# Autodesk Inventor assembly: Milestone 2 Assembly
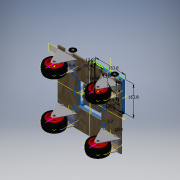
[picture p0: Inventor's stored thumbnail of the model, 180x180]
Saved by Autodesk Inventor 2016 (Build 200138000, 138)
## iProperties
Created: 2016-03-08
Part Number: Milestone 2 Assembly
Document SubType Name: Assembly
Designer: Kenneth Daniel
Author: Kenneth Daniel
## Documents named in this file (38)
- C:\Users\Kenneth Daniel\Documents\Enes 100A\Milestone 2\Milestone 2 Assembly.iam
- C:\Users\Kenneth Daniel\Documents\Enes 100A\Milestone 2\Lifting Platform With Balance.ipt
- C:\Users\Kenneth Daniel\Documents\Enes 100A\Milestone 2\To Much Work, Motor.ipt
- C:\Users\Kenneth Daniel\Documents\Enes 100A\Milestone One\PH Monitor.ipt
- C:\Users\Kenneth Daniel\Documents\Enes 100A\Milestone 2\Lifting Chasis Assembly Milestone 2.iam
- C:\Users\Kenneth Daniel\Documents\Enes 100A\Milestone 2\Lifting Motor Platform.ipt
- C:\Users\Kenneth Daniel\Documents\Enes 100A\Milestone 2\Milestone 2 Main Vehicle Chassis.ipt
- C:\Users\Kenneth Daniel\Documents\Enes 100A\arduino uno.iam
- C:\Users\Kenneth Daniel\Documents\Inventor\Content Center Files\R2016\en-US\AS 1427(00)\AS 1427 - M5 x 20(4).ipt
- C:\Users\Kenneth Daniel\Documents\Enes 100A\Milestone 2\Motors Mount For Chassis.ipt
- C:\Users\Kenneth Daniel\Documents\Enes 100A\CorrectMotor_CAD_spencermical_enes100OSVproject_4-50pm-3-3-16-thursday-freshmanyear-springsemester.ipt
- C:\Users\Kenneth Daniel\Documents\Enes 100A\Milestone 2\Updated Milestone 2 Wheel.ipt
- C:\Users\Kenneth Daniel\Documents\Enes 100A\Milestone 2\Milestone 2 Rim.ipt
- C:\Users\Kenneth Daniel\Documents\Enes 100A\Milestone 2\Small Sprocket.ipt
- C:\Users\Kenneth Daniel\Documents\Enes 100A\Milestone 2\Motors Mount For Chassis_MIR.ipt
- C:\Users\Kenneth Daniel\Documents\Enes 100A\CorrectMotor_CAD_spencermical_enes100OSVproject_4-50pm-3-3-16-thursday-freshmanyear-springsemester_MIR.ipt
- C:\Users\Kenneth Daniel\Documents\Enes 100A\Milestone 2\Motors Mount For Chassis_MIR2.ipt
- C:\Users\Kenneth Daniel\Documents\Enes 100A\CorrectMotor_CAD_spencermical_enes100OSVproject_4-50pm-3-3-16-thursday-freshmanyear-springsemester_MIR2.ipt
- C:\Users\Kenneth Daniel\Documents\Enes 100A\Milestone 2\Motors Mount For Chassis_MIR2_MIR.ipt
- C:\Users\Kenneth Daniel\Documents\Enes 100A\CorrectMotor_CAD_spencermical_enes100OSVproject_4-50pm-3-3-16-thursday-freshmanyear-springsemester_MIR2_MIR.ipt
- C:\Users\Kenneth Daniel\Documents\Enes 100A\Milestone 2\Small Sprocket_MIR.ipt
- C:\Users\Kenneth Daniel\Documents\Enes 100A\Milestone 2\Small Sprocket_MIR1.ipt
- C:\Users\Kenneth Daniel\Documents\Enes 100A\Milestone 2\Small Sprocket_MIR_MIR.ipt
- C:\Users\Kenneth Daniel\Documents\Inventor\Content Center Files\R2016\en-US\CNS 3128\CNS 3128 - M 5 x 0.8.ipt
- C:\Users\Kenneth Daniel\Documents\Enes 100A\Milestone 2\Wheel Holder Milestone 2.ipt
- C:\Users\Kenneth Daniel\Documents\Enes 100A\Milestone 2\Updated Milestone 2 Wheel_MIR6.ipt
- C:\Users\Kenneth Daniel\Documents\Enes 100A\Milestone 2\Milestone 2 Rim_MIR6.ipt
- C:\Users\Kenneth Daniel\Documents\Enes 100A\Milestone 2\Wheel Holder Milestone 2_MIR6.ipt
- C:\Users\Kenneth Daniel\Documents\Enes 100A\Milestone 2\Updated Milestone 2 Wheel_MIR7.ipt
- C:\Users\Kenneth Daniel\Documents\Enes 100A\Milestone 2\Milestone 2 Rim_MIR7.ipt
- C:\Users\Kenneth Daniel\Documents\Enes 100A\Milestone 2\Wheel Holder Milestone 2_MIR7.ipt
- C:\Users\Kenneth Daniel\Documents\Enes 100A\Milestone 2\Updated Milestone 2 Wheel_MIR6_MIR.ipt
- C:\Users\Kenneth Daniel\Documents\Enes 100A\Milestone 2\Milestone 2 Rim_MIR6_MIR.ipt
- C:\Users\Kenneth Daniel\Documents\Enes 100A\Milestone 2\Wheel Holder Milestone 2_MIR6_MIR.ipt
- C:\Users\Kenneth Daniel\Documents\Enes 100A\Simplistic_battery_pack-superdroid-spencermical.ipt
- C:\Users\Kenneth Daniel\Documents\Enes 100A\Syringe_moreaccurate_ENES100_OSV-spencermical-4-52pm-3-5-16-saturday.ipt
- C:\Users\Kenneth Daniel\Documents\Enes 100A\Larger Syringe.ipt
- C:\Users\Kenneth Daniel\Documents\Enes 100A\Vex Motor.iam
## Components (52 placed, 37 different names)
1. Lifting Platform With Balance:1 — Mate:8, Mate:9, Mate:10, Mate:11, Mate:18, Mate:19
2. To Much Work, Motor:1 — Mate:8, Mate:9
3. PH Monitor:1 — Mate:10, Mate:11
4. Lifting Chasis Assembly Milestone 2:1 [sub-assembly] — Mate:15, Mate:16, Mate:17, Mate:18, Mate:19, Mate:20, Mate:21, Mate:22, Mate:90
5. Lifting Motor Platform:1 — Mate:15, Mate:16, Mate:17, Mate:92, Angle:1, Mate:93, Flush:28
6. Milestone 2 Main Vehicle Chassis:1 — Mate:20, Mate:21, Mate:22, Mate:23, Mate:33, Mate:34, Mate:35, Mate:36, Flush:5, Mate:37, Flush:6, Mate:39, Mate:49, Mate:52, Mate:57, Mate:62, Mate:63, Mate:72, Mate:74, Mate:76, Mate:77, Mate:78, Mate:79, Flush:13, Flush:18, Flush:24, Flush:25, Flush:26, Flush:27, Mate:89, Tangent:1, Tangent:2, Mate:94, Mate:95
7. arduino uno:1 [sub-assembly] — Mate:33, Mate:34
8. AS 1427 - Metric M5 x 20:1 — Mate:50, Mate:51, Mate:57, Mate:73
9. AS 1427 - Metric M5 x 20:2 — Mate:55, Mate:56, Mate:71
10. AS 1427 - Metric M5 x 20:3 — Mate:60, Mate:61
11. AS 1427 - Metric M5 x 20:4 — Mate:58, Mate:59, Mate:62
12. AS 1427 - Metric M5 x 20:5 — Mate:53, Mate:54
13. AS 1427 - Metric M5 x 20:8 — Mate:47, Mate:48, Mate:49, Mate:75
14. Motors Mount For Chassis:1 — Mate:31, Mate:37, Mate:38, Mate:53, Mate:54, Mate:55, Mate:56
15. CorrectMotor_CAD_spencermical_enes100OSVproject_4-50pm-3-3-16-thursday-freshmanyear-springsemester:4 — Mate:31, Mate:38, Flush:6, Mate:39
16. Updated Milestone 2 Wheel:1 — Mate:24, Flush:1
17. Milestone 2 Rim:4 — Mate:24, Flush:1, Mate:80, Mate:81
18. Small Sprocket:5 — Flush:7, Mate:70
19. Motors Mount For Chassis_MIR:1 — Mate:40, Mate:41, Mate:47, Mate:48, Mate:50, Mate:51, Mate:52
20. CorrectMotor_CAD_spencermical_enes100OSVproject_4-50pm-3-3-16-thursday-freshmanyear-springsemester_MIR:1 — Mate:40, Mate:41
21. Motors Mount For Chassis_MIR2:1 — Mate:42, Mate:43, Mate:58, Mate:59, Mate:60, Mate:61, Mate:63
22. CorrectMotor_CAD_spencermical_enes100OSVproject_4-50pm-3-3-16-thursday-freshmanyear-springsemester_MIR2:1 — Mate:42, Mate:43
23. AS 1427 - Metric M5 x 20:9 — Mate:64, Mate:65
24. AS 1427 - Metric M5 x 20:10 — Mate:66, Mate:67
25. Motors Mount For Chassis_MIR2_MIR:1 — Mate:64, Mate:65, Mate:66, Mate:67, Mate:68, Mate:69
26. CorrectMotor_CAD_spencermical_enes100OSVproject_4-50pm-3-3-16-thursday-freshmanyear-springsemester_MIR2_MIR:1 — Mate:68, Mate:69, Flush:7, Mate:70
27. Small Sprocket_MIR:1
28. Small Sprocket_MIR1:1
29. Small Sprocket_MIR_MIR:1
30. CNS 3128 M 5:1 — Mate:75, Mate:76
31. CNS 3128 M 5:2 — Mate:71, Mate:72
32. CNS 3128 M 5:4 — Mate:73, Mate:74
33. CNS 3128 M 5:5
34. CNS 3128 M 5:6
35. CNS 3128 M 5:7
36. CNS 3128 M 5:8
37. CNS 3128 M 5:9
38. Wheel Holder Milestone 2:2 — Mate:77, Mate:78, Mate:79, Mate:80, Mate:81, Flush:13, Flush:18, Flush:27
39. Updated Milestone 2 Wheel_MIR6:1 — Flush:19, Mate:82
40. Milestone 2 Rim_MIR6:1 — Flush:19, Mate:82, Flush:20, Mate:83
41. Wheel Holder Milestone 2_MIR6:1 — Flush:20, Mate:83, Flush:25
42. Updated Milestone 2 Wheel_MIR7:1 — Flush:21, Mate:84
43. Milestone 2 Rim_MIR7:1 — Flush:21, Mate:84, Flush:22, Mate:85
44. Wheel Holder Milestone 2_MIR7:1 — Flush:22, Mate:85, Flush:26
45. Updated Milestone 2 Wheel_MIR6_MIR:1 — Mate:86, Flush:23
46. Milestone 2 Rim_MIR6_MIR:1 — Mate:86, Flush:23, Mate:87, Mate:88
47. Wheel Holder Milestone 2_MIR6_MIR:1 — Mate:87, Mate:88, Flush:24
48. Simplistic_battery_pack-superdroid-spencermical:1 — Mate:89, Mate:90
49. Syringe_moreaccurate_ENES100_OSV-spencermical-4-52pm-3-5-16-saturday:2 — Mate:91, Tangent:1
50. Larger Syringe:1 — Tangent:2
51. Vex Motor:1 [sub-assembly] — Mate:92, Angle:1, Mate:93, Flush:28
52. Vex Motor:2 [sub-assembly] — Mate:94, Mate:95
## Relationships (94: Mate 75, Flush 16, Tangent 2, Angle 1)
- Mate:8: Lifting Platform With Balance:1 ↔ To Much Work, Motor:1
- Mate:9: Lifting Platform With Balance:1 ↔ To Much Work, Motor:1
- Mate:10: Lifting Platform With Balance:1 ↔ PH Monitor:1
- Mate:11: Lifting Platform With Balance:1 ↔ PH Monitor:1
- Mate:15: Lifting Chasis Assembly Milestone 2:1 ↔ Lifting Motor Platform:1
- Mate:16: Lifting Chasis Assembly Milestone 2:1 ↔ Lifting Motor Platform:1
- Mate:17: Lifting Chasis Assembly Milestone 2:1 ↔ Lifting Motor Platform:1
- Mate:18 (20.1 mm): Lifting Platform With Balance:1 ↔ Lifting Chasis Assembly Milestone 2:1
- Mate:19 (20.1 mm): Lifting Platform With Balance:1 ↔ Lifting Chasis Assembly Milestone 2:1
- Mate:20: Lifting Chasis Assembly Milestone 2:1 ↔ Milestone 2 Main Vehicle Chassis:1
- Mate:21: Lifting Chasis Assembly Milestone 2:1 ↔ Milestone 2 Main Vehicle Chassis:1
- Mate:22: Lifting Chasis Assembly Milestone 2:1 ↔ Milestone 2 Main Vehicle Chassis:1
- Mate:23: Milestone 2 Main Vehicle Chassis:1
- Mate:24: Updated Milestone 2 Wheel:1 ↔ Milestone 2 Rim:4
- Flush:1: Updated Milestone 2 Wheel:1 ↔ Milestone 2 Rim:4
- Mate:31: Motors Mount For Chassis:1 ↔ CorrectMotor_CAD_spencermical_enes100OSVproject_4-50pm-3-3-16-thursday-freshmanyear-springsemester:4
- Mate:33: Milestone 2 Main Vehicle Chassis:1 ↔ arduino uno:1
- Mate:34: Milestone 2 Main Vehicle Chassis:1 ↔ arduino uno:1
- Mate:35: Milestone 2 Main Vehicle Chassis:1
- Mate:36: Milestone 2 Main Vehicle Chassis:1
- Flush:5: Milestone 2 Main Vehicle Chassis:1
- Mate:37: Milestone 2 Main Vehicle Chassis:1 ↔ Motors Mount For Chassis:1
- Mate:38 (-25 mm): Motors Mount For Chassis:1 ↔ CorrectMotor_CAD_spencermical_enes100OSVproject_4-50pm-3-3-16-thursday-freshmanyear-springsemester:4
- Flush:6 (-10.294 mm): Milestone 2 Main Vehicle Chassis:1 ↔ CorrectMotor_CAD_spencermical_enes100OSVproject_4-50pm-3-3-16-thursday-freshmanyear-springsemester:4
- Mate:39 (-58.5 mm): Milestone 2 Main Vehicle Chassis:1 ↔ CorrectMotor_CAD_spencermical_enes100OSVproject_4-50pm-3-3-16-thursday-freshmanyear-springsemester:4
- Mate:40 (-25 mm): Motors Mount For Chassis_MIR:1 ↔ CorrectMotor_CAD_spencermical_enes100OSVproject_4-50pm-3-3-16-thursday-freshmanyear-springsemester_MIR:1
- Mate:41: Motors Mount For Chassis_MIR:1 ↔ CorrectMotor_CAD_spencermical_enes100OSVproject_4-50pm-3-3-16-thursday-freshmanyear-springsemester_MIR:1
- Mate:42 (-25 mm): Motors Mount For Chassis_MIR2:1 ↔ CorrectMotor_CAD_spencermical_enes100OSVproject_4-50pm-3-3-16-thursday-freshmanyear-springsemester_MIR2:1
- Mate:43: Motors Mount For Chassis_MIR2:1 ↔ CorrectMotor_CAD_spencermical_enes100OSVproject_4-50pm-3-3-16-thursday-freshmanyear-springsemester_MIR2:1
- Mate:47: AS 1427 - Metric M5 x 20:8 ↔ Motors Mount For Chassis_MIR:1
- Mate:48: AS 1427 - Metric M5 x 20:8 ↔ Motors Mount For Chassis_MIR:1
- Mate:49: Milestone 2 Main Vehicle Chassis:1 ↔ AS 1427 - Metric M5 x 20:8
- Mate:50: AS 1427 - Metric M5 x 20:1 ↔ Motors Mount For Chassis_MIR:1
- Mate:51: AS 1427 - Metric M5 x 20:1 ↔ Motors Mount For Chassis_MIR:1
- Mate:52: Milestone 2 Main Vehicle Chassis:1 ↔ Motors Mount For Chassis_MIR:1
- Mate:53: AS 1427 - Metric M5 x 20:5 ↔ Motors Mount For Chassis:1
- Mate:54: AS 1427 - Metric M5 x 20:5 ↔ Motors Mount For Chassis:1
- Mate:55: AS 1427 - Metric M5 x 20:2 ↔ Motors Mount For Chassis:1
- Mate:56: AS 1427 - Metric M5 x 20:2 ↔ Motors Mount For Chassis:1
- Mate:57: Milestone 2 Main Vehicle Chassis:1 ↔ AS 1427 - Metric M5 x 20:1
- Mate:58: AS 1427 - Metric M5 x 20:4 ↔ Motors Mount For Chassis_MIR2:1
- Mate:59: AS 1427 - Metric M5 x 20:4 ↔ Motors Mount For Chassis_MIR2:1
- Mate:60: AS 1427 - Metric M5 x 20:3 ↔ Motors Mount For Chassis_MIR2:1
- Mate:61: AS 1427 - Metric M5 x 20:3 ↔ Motors Mount For Chassis_MIR2:1
- Mate:62: Milestone 2 Main Vehicle Chassis:1 ↔ AS 1427 - Metric M5 x 20:4
- Mate:63: Milestone 2 Main Vehicle Chassis:1 ↔ Motors Mount For Chassis_MIR2:1
- Mate:64: AS 1427 - Metric M5 x 20:9 ↔ Motors Mount For Chassis_MIR2_MIR:1
- Mate:65: AS 1427 - Metric M5 x 20:9 ↔ Motors Mount For Chassis_MIR2_MIR:1
- Mate:66: AS 1427 - Metric M5 x 20:10 ↔ Motors Mount For Chassis_MIR2_MIR:1
- Mate:67: AS 1427 - Metric M5 x 20:10 ↔ Motors Mount For Chassis_MIR2_MIR:1
- Mate:68: Motors Mount For Chassis_MIR2_MIR:1 ↔ CorrectMotor_CAD_spencermical_enes100OSVproject_4-50pm-3-3-16-thursday-freshmanyear-springsemester_MIR2_MIR:1
- Mate:69 (-25 mm): Motors Mount For Chassis_MIR2_MIR:1 ↔ CorrectMotor_CAD_spencermical_enes100OSVproject_4-50pm-3-3-16-thursday-freshmanyear-springsemester_MIR2_MIR:1
- Flush:7: Small Sprocket:5 ↔ CorrectMotor_CAD_spencermical_enes100OSVproject_4-50pm-3-3-16-thursday-freshmanyear-springsemester_MIR2_MIR:1
- Mate:70: Small Sprocket:5 ↔ CorrectMotor_CAD_spencermical_enes100OSVproject_4-50pm-3-3-16-thursday-freshmanyear-springsemester_MIR2_MIR:1
- Mate:71: AS 1427 - Metric M5 x 20:2 ↔ CNS 3128 M 5:2
- Mate:72: Milestone 2 Main Vehicle Chassis:1 ↔ CNS 3128 M 5:2
- Mate:73: AS 1427 - Metric M5 x 20:1 ↔ CNS 3128 M 5:4
- Mate:74: Milestone 2 Main Vehicle Chassis:1 ↔ CNS 3128 M 5:4
- Mate:75: AS 1427 - Metric M5 x 20:8 ↔ CNS 3128 M 5:1
- Mate:76: Milestone 2 Main Vehicle Chassis:1 ↔ CNS 3128 M 5:1
- Mate:77: Milestone 2 Main Vehicle Chassis:1 ↔ Wheel Holder Milestone 2:2
- Mate:78: Milestone 2 Main Vehicle Chassis:1 ↔ Wheel Holder Milestone 2:2
- Mate:79: Milestone 2 Main Vehicle Chassis:1 ↔ Wheel Holder Milestone 2:2
- Mate:80: Milestone 2 Rim:4 ↔ Wheel Holder Milestone 2:2
- Mate:81 (-22 mm): Milestone 2 Rim:4 ↔ Wheel Holder Milestone 2:2
- Flush:13: Milestone 2 Main Vehicle Chassis:1 ↔ Wheel Holder Milestone 2:2
- Flush:18: Milestone 2 Main Vehicle Chassis:1 ↔ Wheel Holder Milestone 2:2
- Flush:19: Updated Milestone 2 Wheel_MIR6:1 ↔ Milestone 2 Rim_MIR6:1
- Mate:82: Updated Milestone 2 Wheel_MIR6:1 ↔ Milestone 2 Rim_MIR6:1
- Flush:20 (-22 mm): Milestone 2 Rim_MIR6:1 ↔ Wheel Holder Milestone 2_MIR6:1
- Mate:83: Milestone 2 Rim_MIR6:1 ↔ Wheel Holder Milestone 2_MIR6:1
- Flush:21: Updated Milestone 2 Wheel_MIR7:1 ↔ Milestone 2 Rim_MIR7:1
- Mate:84: Updated Milestone 2 Wheel_MIR7:1 ↔ Milestone 2 Rim_MIR7:1
- Flush:22 (-22 mm): Milestone 2 Rim_MIR7:1 ↔ Wheel Holder Milestone 2_MIR7:1
- Mate:85: Milestone 2 Rim_MIR7:1 ↔ Wheel Holder Milestone 2_MIR7:1
- Mate:86: Updated Milestone 2 Wheel_MIR6_MIR:1 ↔ Milestone 2 Rim_MIR6_MIR:1
- Flush:23: Updated Milestone 2 Wheel_MIR6_MIR:1 ↔ Milestone 2 Rim_MIR6_MIR:1
- Mate:87: Milestone 2 Rim_MIR6_MIR:1 ↔ Wheel Holder Milestone 2_MIR6_MIR:1
- Mate:88 (-22 mm): Milestone 2 Rim_MIR6_MIR:1 ↔ Wheel Holder Milestone 2_MIR6_MIR:1
- Flush:24: Milestone 2 Main Vehicle Chassis:1 ↔ Wheel Holder Milestone 2_MIR6_MIR:1
- Flush:25: Milestone 2 Main Vehicle Chassis:1 ↔ Wheel Holder Milestone 2_MIR6:1
- Flush:26: Milestone 2 Main Vehicle Chassis:1 ↔ Wheel Holder Milestone 2_MIR7:1
- Flush:27: Milestone 2 Main Vehicle Chassis:1 ↔ Wheel Holder Milestone 2:2
- Mate:89: Milestone 2 Main Vehicle Chassis:1 ↔ Simplistic_battery_pack-superdroid-spencermical:1
- Mate:90 (15 mm): Lifting Chasis Assembly Milestone 2:1 ↔ Simplistic_battery_pack-superdroid-spencermical:1
- Mate:91: Syringe_moreaccurate_ENES100_OSV-spencermical-4-52pm-3-5-16-saturday:2
- Tangent:1: Milestone 2 Main Vehicle Chassis:1 ↔ Syringe_moreaccurate_ENES100_OSV-spencermical-4-52pm-3-5-16-saturday:2
- Tangent:2: Milestone 2 Main Vehicle Chassis:1 ↔ Larger Syringe:1
- Mate:92: Lifting Motor Platform:1 ↔ Vex Motor:1
- Angle:1 (0 deg): Lifting Motor Platform:1 ↔ Vex Motor:1
- Mate:93 (-1.8455 mm): Lifting Motor Platform:1 ↔ Vex Motor:1
- Flush:28 (59.39 mm): Lifting Motor Platform:1 ↔ Vex Motor:1
- Mate:94: Milestone 2 Main Vehicle Chassis:1 ↔ Vex Motor:2
- Mate:95: Milestone 2 Main Vehicle Chassis:1 ↔ Vex Motor:2
